# Autodesk Inventor assembly: board2.brd
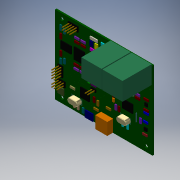
[picture p0: Inventor's stored thumbnail of the model, 180x180]
Saved by Autodesk Inventor 2016 (Build 200138000, 138)
## iProperties
Created: 2016-04-08
Part Number: board2.brd
Document SubType Name: Assembly
Designer: Paschalis
Author: Paschalis
## Documents named in this file (48)
- C:\Users\Paschalis\Documents\eagle\Measuring-PCB\3D\New3DTry\board2.brd.iam
- C:\Users\Paschalis\Documents\eagle\Measuring-PCB\3D\New3DTry\board2.brd_Outline.ipt
- C:\Users\Paschalis\Documents\eagle\Measuring-PCB\3D\New3DTry\PHOENIX-TERMINAL-3PIN, PHOENIX-TERMINAL-3PIN_1.ipt
- C:\Users\Paschalis\Documents\eagle\Measuring-PCB\3D\New3DTry\SOT95P280X145-6N, ADR3425ARJZ-R7_3.ipt
- C:\Users\Paschalis\Documents\eagle\Measuring-PCB\3D\New3DTry\SOP65P780X200-28N, ADS1256IDBT_5.ipt
- C:\Users\Paschalis\Documents\eagle\Measuring-PCB\3D\New3DTry\SOIC127P1032X265-16N, ADUM5000ARWZ_7.ipt
- C:\Users\Paschalis\Documents\eagle\Measuring-PCB\3D\New3DTry\1X02_NO_SILK, AIN6-7_1X02_NO_SILK_9.ipt
- C:\Users\Paschalis\Documents\eagle\Measuring-PCB\3D\New3DTry\TQFP32-08, ATMEGA328P_TQFP_11.ipt
- C:\Users\Paschalis\Documents\eagle\Measuring-PCB\3D\New3DTry\BATTCON_12MM, 3V_13.ipt
- C:\Users\Paschalis\Documents\eagle\Measuring-PCB\3D\New3DTry\C3216, 10U_15.ipt
- C:\Users\Paschalis\Documents\eagle\Measuring-PCB\3D\New3DTry\C3216, 0_1U_17.ipt
- C:\Users\Paschalis\Documents\eagle\Measuring-PCB\3D\New3DTry\C3216, 47U_19.ipt
- C:\Users\Paschalis\Documents\eagle\Measuring-PCB\3D\New3DTry\C3216, 100P_22.ipt
- C:\Users\Paschalis\Documents\eagle\Measuring-PCB\3D\New3DTry\C3216, 18P_26.ipt
- C:\Users\Paschalis\Documents\eagle\Measuring-PCB\3D\New3DTry\C3216, 1U_47.ipt
- C:\Users\Paschalis\Documents\eagle\Measuring-PCB\3D\New3DTry\C3216, 10N_49.ipt
- C:\Users\Paschalis\Documents\eagle\Measuring-PCB\3D\New3DTry\C3216, 2_2U_51.ipt
- C:\Users\Paschalis\Documents\eagle\Measuring-PCB\3D\New3DTry\C3216, 22P_53.ipt
- C:\Users\Paschalis\Documents\eagle\Measuring-PCB\3D\New3DTry\1X04_NO_SILK_ALL_ROUND, D0-D3_1X04_NO_SILK_ALL_ROUND_59.ipt
- C:\Users\Paschalis\Documents\eagle\Measuring-PCB\3D\New3DTry\DS3234, DS3234_61.ipt
- C:\Users\Paschalis\Documents\eagle\Measuring-PCB\3D\New3DTry\PAS_5X20, 15A_63.ipt
- C:\Users\Paschalis\Documents\eagle\Measuring-PCB\3D\New3DTry\2X3, FEMALE_65.ipt
- C:\Users\Paschalis\Documents\eagle\Measuring-PCB\3D\New3DTry\2X04, ISOLATED_CON_2X04_67.ipt
- C:\Users\Paschalis\Documents\eagle\Measuring-PCB\3D\New3DTry\1X03, JP1A_1X03_69.ipt
- C:\Users\Paschalis\Documents\eagle\Measuring-PCB\3D\New3DTry\1X03, JP1B_1X03_71.ipt
- C:\Users\Paschalis\Documents\eagle\Measuring-PCB\3D\New3DTry\1X03, JP2A_1X03_73.ipt
- C:\Users\Paschalis\Documents\eagle\Measuring-PCB\3D\New3DTry\1X03, JP2B_1X03_75.ipt
- C:\Users\Paschalis\Documents\eagle\Measuring-PCB\3D\New3DTry\CHIPLED_0805, LED1_CHIPLED_0805_77.ipt
- C:\Users\Paschalis\Documents\eagle\Measuring-PCB\3D\New3DTry\SOT95P280X145-5N, LP2985-33DBVT_79.ipt
- C:\Users\Paschalis\Documents\eagle\Measuring-PCB\3D\New3DTry\SOIC-16, IC_DIL16-SOIC-16_81.ipt
- C:\Users\Paschalis\Documents\eagle\Measuring-PCB\3D\New3DTry\2X04, NON-ISOLATED_CON_2X04_83.ipt
- C:\Users\Paschalis\Documents\eagle\Measuring-PCB\3D\New3DTry\HC49U-V, 7_68MHZ_85.ipt
- C:\Users\Paschalis\Documents\eagle\Measuring-PCB\3D\New3DTry\HC49U-V, 16MHZ_87.ipt
- C:\Users\Paschalis\Documents\eagle\Measuring-PCB\3D\New3DTry\LVK25, 0_005_89.ipt
- C:\Users\Paschalis\Documents\eagle\Measuring-PCB\3D\New3DTry\R3216, 4_7K_91.ipt
- C:\Users\Paschalis\Documents\eagle\Measuring-PCB\3D\New3DTry\M3216, 560K_93.ipt
- C:\Users\Paschalis\Documents\eagle\Measuring-PCB\3D\New3DTry\M3216, 5_49M_95.ipt
- C:\Users\Paschalis\Documents\eagle\Measuring-PCB\3D\New3DTry\M3216, 1K_100.ipt
- C:\Users\Paschalis\Documents\eagle\Measuring-PCB\3D\New3DTry\R3216, 100_105.ipt
- C:\Users\Paschalis\Documents\eagle\Measuring-PCB\3D\New3DTry\R3216, 10K_109.ipt
- C:\Users\Paschalis\Documents\eagle\Measuring-PCB\3D\New3DTry\R3216, 1K_113.ipt
- C:\Users\Paschalis\Documents\eagle\Measuring-PCB\3D\New3DTry\TACTILE_SWITCH_TALL, SWITCH-MOMENTARY-2SMD-4_115.ipt
- C:\Users\Paschalis\Documents\eagle\Measuring-PCB\3D\New3DTry\SJ, RST_SJ_117.ipt
- C:\Users\Paschalis\Documents\eagle\Measuring-PCB\3D\New3DTry\1X02, RX-TX_1X02_119.ipt
- C:\Users\Paschalis\Documents\eagle\Measuring-PCB\3D\New3DTry\SJ, SYNC_SJ_121.ipt
- C:\Users\Paschalis\Documents\eagle\Measuring-PCB\3D\New3DTry\PAS-PHOENIXTERMINAL-2PIN-10_16MM, PAS-PHOENIXTERMINAL2PIN-10_16MM_123.ipt
- C:\Users\Paschalis\Documents\eagle\Measuring-PCB\3D\headers.ipt
- C:\Users\Paschalis\Documents\eagle\Measuring-PCB\3D\crystals.ipt
## Components (84 placed, 84 different names)
1. board2.brd_Outline:1 — Flush:2, Flush:4
2. 1WIRE-BUS_2
3. ADR3425_4
4. ADS1256_6
5. ADUM5000_8
6. AIN6-7_10
7. ATMEGA328_12
8. BAT1_14
9. C1_16
10. C2_18
11. C3_20
12. C4_21
13. C5_23
14. C6_24
15. C7_25
16. C8_27
17. C9_28
18. C10_29
19. C11_30
20. C12_31
21. C13_32
22. C14_33
23. C15_34
24. C16_35
25. C17_36
26. C18_37
27. C19_38
28. C20_39
29. C21_40
30. C22_41
31. C23_42
32. C24_43
33. C25_44
34. C26_45
35. C27_46
36. C28_48
37. C29_50
38. C30_52
39. C31_54
40. C32_55
41. C33_56
42. C34_57
43. C35_58
44. D0-D3_60
45. DS3234_62
46. F1_64
47. 2X3_66
48. ISOLATED_CON_68 — Flush:1
49. JP1A_70
50. JP1B_72
51. JP2A_74
52. JP2B_76
53. LED1_78
54. LP2985_80
55. MAX14850_82
56. NON-ISOLATED_CON_84
57. Q1_86
58. Q2_88 — Flush:3
59. R1_90
60. R2_92
61. R2A40_94
62. R2A400_96
63. R2B40_97
64. R2B400_98
65. R3_99
66. R3A_101
67. R3B_102
68. R4_103
69. R5_104
70. R6_106
71. R7_107
72. R8_108
73. R9_110
74. R10_111
75. R11_112
76. R12_114
77. RESET_116
78. RST_118
79. RX-TX_120
80. SYNC_122
81. VOUT_124
82. VPANEL_125
83. headers:1 — Flush:1, Flush:2
84. crystals:1 — Flush:3, Flush:4
## Relationships (4: Flush 4)
- Flush:1: ISOLATED_CON_68 ↔ headers:1
- Flush:2: board2.brd_Outline:1 ↔ headers:1
- Flush:3: Q2_88 ↔ crystals:1
- Flush:4: board2.brd_Outline:1 ↔ crystals:1
